# Autodesk Inventor assembly: __VK_WT_ZSB
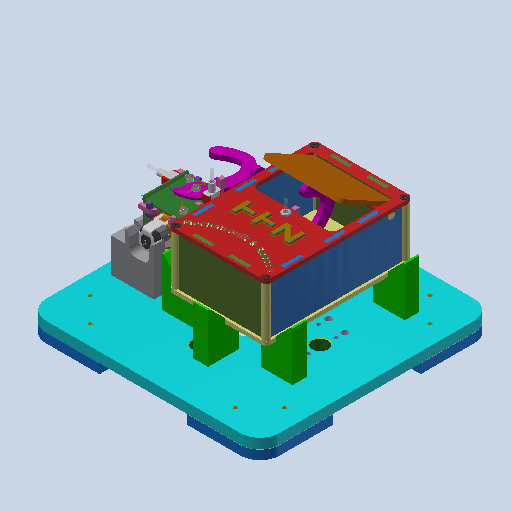
[picture p0: Inventor's stored thumbnail of the model, 512x512]
Saved by Autodesk Inventor 2025.1 (Build 291241000, 241)
## iProperties
Created: 2023-11-18
Part Number: __VK_WT_ZSB
Material: Generisch
Document SubType Name: Assembly
Designer: RP
Author: RP
## Documents named in this file (4)
- C:\Users\Erik\Erik\Hochschule\3. Semester\CAD\CAD-Paspa\Useless Box\_Verkettung\__VK_WT_beladen.iam
- C:\Users\Erik\Erik\Hochschule\3. Semester\CAD\CAD-Paspa\Useless Box\_Verkettung\__VK_WT.iam
- C:\Users\Erik\Erik\Hochschule\3. Semester\CAD\CAD-Paspa\Useless Box\_Useless_Box\Useless_Box.iam
- C:\Users\Erik\Erik\Hochschule\3. Semester\CAD\CAD-Paspa\Useless Box\_Useless_Box\Antriebseinheit_ZSB.iam
## Components (4 placed, 3 different names)
1. __VK_WT:1 [sub-assembly] — Flush:16, Flush:17, Flush:18, Mate:12
2. Useless_Box:1 [sub-assembly] — Mate:12, Flush:28
3. Antriebseinheit_ZSB:1 [sub-assembly] — Flush:28
4. Antriebseinheit_ZSB:2 [sub-assembly]
## Relationships (20: Mate 15, Flush 5)
- [Flush]: __VK_WT:1
- [Mate]: __VK_WT:1
- [Mate] (20.3 mm): __VK_WT:1
- Flush:16: __VK_WT:1
- Flush:17: __VK_WT:1
- Flush:18: __VK_WT:1
- [Mate]: __VK_WT:1 ↔ Useless_Box:1
- [Mate]: __VK_WT:1 ↔ Useless_Box:1
- Mate:12: __VK_WT:1 ↔ Useless_Box:1
- [Mate]: __VK_WT:1 ↔ Antriebseinheit_ZSB:1
- [Mate]: __VK_WT:1 ↔ Antriebseinheit_ZSB:1
- [Mate]: __VK_WT:1 ↔ Antriebseinheit_ZSB:1
- [Mate]: __VK_WT:1 ↔ Antriebseinheit_ZSB:2
- [Mate]: __VK_WT:1 ↔ Antriebseinheit_ZSB:2
- [Mate]: __VK_WT:1 ↔ Antriebseinheit_ZSB:2
- [Mate]: __VK_WT:1 ↔ Antriebseinheit_ZSB:1
- [Mate]: __VK_WT:1 ↔ Antriebseinheit_ZSB:1
- [Mate]: __VK_WT:1 ↔ Antriebseinheit_ZSB:1
- [Mate]: __VK_WT:1 ↔ Antriebseinheit_ZSB:1
- Flush:28: Useless_Box:1 ↔ Antriebseinheit_ZSB:1
